# Autodesk Inventor assembly: Body
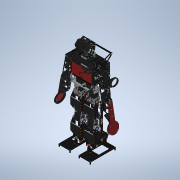
[picture p0: Inventor's stored thumbnail of the model, 180x180]
Saved by Autodesk Inventor 2020.4 (Build 244396000, 396)
## iProperties
Created: 2021-09-30
Part Number: Body
Document SubType Name: Assembly
Designer: Masato Kubotera
Mass: 3701.21 g
Surface Area: 13379.4 cm^2
Volume: 3277.75 cm^3
Density: 1.12919 g/cm^3
Author: Masato Kubotera
## Documents named in this file (4)
- C:\Users\Masato\Desktop\SUSTAINA-OP\Body.iam
- C:\Users\Masato\Desktop\SUSTAINA-OP\UpperBody\UpperBody.iam
- C:\Users\Masato\Desktop\SUSTAINA-OP\LowerBody\LowerBody.iam
- C:\Users\Masato\Desktop\SUSTAINA-OP\LowerBody\LowerBody_MIR.iam
## Components (3 placed, 3 different names)
1. UpperBody:1 [sub-assembly] — フラッシュ:1, 挿入:2, 挿入:3
2. LowerBody_MIR:1 [sub-assembly] — 挿入:2
3. LowerBody:1 [sub-assembly] — 挿入:3
## Relationships (3: Insert 2, Flush 1)
- フラッシュ:1 [Flush]: UpperBody:1
- 挿入:2 [Insert]: UpperBody:1 ↔ LowerBody_MIR:1
- 挿入:3 [Insert]: UpperBody:1 ↔ LowerBody:1
